# Autodesk Inventor assembly: kolo_przednie
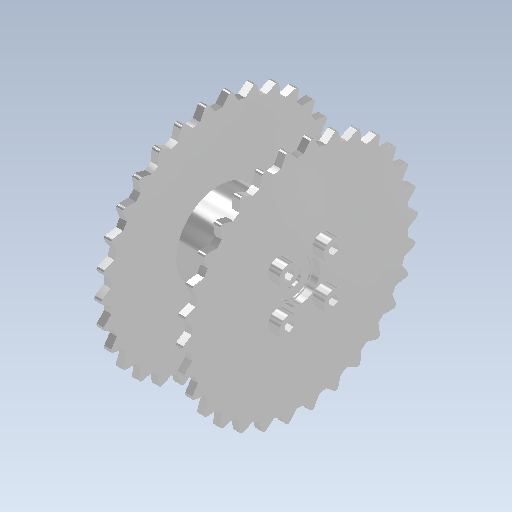
[picture p0: Inventor's stored thumbnail of the model, 512x512]
Saved by Autodesk Inventor 2020.3 (Build 243373000, 373)
## iProperties
Created: 2021-04-05
Part Number: kolo_przednie
Document SubType Name: Assembly
Designer: patry
Mass: 114.8 g
Surface Area: 310.048 cm^2
Volume: 42.5185 cm^3
Density: 2.7 g/cm^3
Author: patry
## Documents named in this file (6)
- C:\Users\patry\Desktop\Konar staff\Ariadna2.1\ariadna_mechanika\Obszar roboczy\Naped\Kola\kolo_przednie.iam
- C:\Users\patry\Desktop\Konar staff\Ariadna2.1\ariadna_mechanika\Obszar roboczy\Naped\Kola\piasta_kola_przedniego_fi6.ipt
- C:\Users\patry\Desktop\Konar staff\Ariadna2.1\ariadna_mechanika\Obszar roboczy\Naped\Lozyska\686_6mm_13mm_bearing\686_bearing.ipt
- C:\Users\patry\Desktop\Konar staff\Ariadna2.1\ariadna_mechanika\Obszar roboczy\Naped\Sruby\M4_nut_3mm.ipt
- C:\Users\patry\Desktop\Konar staff\Ariadna2.1\ariadna_mechanika\Obszar roboczy\Naped\Sruby\M4x35.ipt
- C:\Users\patry\Desktop\Konar staff\Ariadna2.1\ariadna_mechanika\Obszar roboczy\Naped\Kola\kolo_zebate_duze_fi8_V2.ipt
## Components (13 placed, 5 different names)
1. piasta_kola_przedniego_fi6:1 — Zestawiające:7, Zestawiające:8, Zestawiające:9, Zestawiające:10, Zestawiające:28, Zestawiające:31
2. 686_bearing:1 — Zestawiające:7, Zestawiające:8, Zestawiające:33
3. 686_bearing:2 — Zestawiające:9, Zestawiające:10, Zestawiające:30
4. M4_nut_3mm:1 — Zestawiające:18, Zestawiające:19
5. M4x35:1 — Zestawiające:18, Zestawiające:19, Zestawiające:32, Zestawiające:35
6. M4_nut_3mm:2
7. M4x35:2 — Zestawiające:29, Zestawiające:34
8. M4_nut_3mm:3
9. M4x35:3 — Zestawiające:36, Zestawiające:37
10. M4_nut_3mm:4 — Zestawiające:39
11. M4x35:4 — Zestawiające:38
12. kolo_zebate_duze_fi8_V2:1 — Zestawiające:31, Zestawiające:32, Zestawiające:33, Zestawiające:34, Zestawiające:35, Zestawiające:36, Zestawiające:37, Zestawiające:38
13. kolo_zebate_duze_fi8_V2:2 — Zestawiające:28, Zestawiające:29, Zestawiające:30, Zestawiające:39
## Relationships (24: Mate 24)
- Zestawiające:7 [Mate]: piasta_kola_przedniego_fi6:1 ↔ 686_bearing:1
- Zestawiające:8 [Mate]: piasta_kola_przedniego_fi6:1 ↔ 686_bearing:1
- Zestawiające:9 [Mate]: piasta_kola_przedniego_fi6:1 ↔ 686_bearing:2
- Zestawiające:10 [Mate]: piasta_kola_przedniego_fi6:1 ↔ 686_bearing:2
- Zestawiające:18 [Mate]: M4_nut_3mm:1 ↔ M4x35:1
- Zestawiające:19 [Mate] (-4 mm): M4_nut_3mm:1 ↔ M4x35:1
- [Mate]: M4_nut_3mm:2 ↔ M4x35:2
- [Mate] (-4 mm): M4_nut_3mm:2 ↔ M4x35:2
- [Mate]: M4_nut_3mm:3 ↔ M4x35:3
- [Mate] (-4 mm): M4_nut_3mm:3 ↔ M4x35:3
- [Mate]: M4_nut_3mm:4 ↔ M4x35:4
- [Mate] (-4 mm): M4_nut_3mm:4 ↔ M4x35:4
- Zestawiające:28 [Mate]: piasta_kola_przedniego_fi6:1 ↔ kolo_zebate_duze_fi8_V2:2
- Zestawiające:29 [Mate]: M4x35:2 ↔ kolo_zebate_duze_fi8_V2:2
- Zestawiające:30 [Mate]: 686_bearing:2 ↔ kolo_zebate_duze_fi8_V2:2
- Zestawiające:31 [Mate]: piasta_kola_przedniego_fi6:1 ↔ kolo_zebate_duze_fi8_V2:1
- Zestawiające:32 [Mate]: M4x35:1 ↔ kolo_zebate_duze_fi8_V2:1
- Zestawiające:33 [Mate]: 686_bearing:1 ↔ kolo_zebate_duze_fi8_V2:1
- Zestawiające:34 [Mate]: M4x35:2 ↔ kolo_zebate_duze_fi8_V2:1
- Zestawiające:35 [Mate]: M4x35:1 ↔ kolo_zebate_duze_fi8_V2:1
- Zestawiające:36 [Mate]: M4x35:3 ↔ kolo_zebate_duze_fi8_V2:1
- Zestawiające:37 [Mate]: M4x35:3 ↔ kolo_zebate_duze_fi8_V2:1
- Zestawiające:38 [Mate]: M4x35:4 ↔ kolo_zebate_duze_fi8_V2:1
- Zestawiające:39 [Mate]: M4_nut_3mm:4 ↔ kolo_zebate_duze_fi8_V2:2
## Named parameters: d22_d18 = 0 mm, d23_d19 = -4 mm, d24_d18 = 0 mm, d25_d19 = -4 mm, d26_d18 = 0 mm, d27_d19 = -4 mm
